# Autodesk Inventor assembly: Control Board Assembly
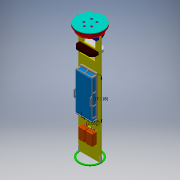
[picture p0: Inventor's stored thumbnail of the model, 180x180]
Saved by Autodesk Inventor 2016 (Build 200138000, 138)
## iProperties
Created: 2017-10-10
Part Number: Control Board Assembly
Document SubType Name: Assembly
Designer: Student
Author: Student
## Documents named in this file (21)
- C:\Users\Student\Documents\Derek Code and Projects\Autodesk\Control Board Assembly.iam
- C:\Users\Student\Documents\Derek Code and Projects\Autodesk\Control board Holder.ipt
- C:\Users\Student\Documents\Derek Code and Projects\Autodesk\Control Board.ipt
- C:\Users\Student\Documents\Derek Code and Projects\Autodesk\Control board Ring Holder.ipt
- C:\Users\Student\Documents\Derek Code and Projects\Autodesk\THE ACTUAL BACK O-RONG FITTING Connection to control board.ipt
- C:\Users\Student\Documents\Derek Code and Projects\Autodesk\Camera Mount.ipt
- C:\Users\Student\Documents\Derek Code and Projects\Autodesk\Camera.ipt
- C:\Users\Student\Documents\Derek Code and Projects\Autodesk\RPI.ipt
- C:\Users\Student\Documents\Derek Code and Projects\Autodesk\Arduino board with Sheild.ipt
- C:\Users\Student\Documents\Derek Code and Projects\Autodesk\Battery.ipt
- C:\Users\Student\Documents\Derek Code and Projects\Autodesk\Voltage Divider (Rough).ipt
- C:\Users\Student\Documents\Derek Code and Projects\Autodesk\Back Lens.ipt
- C:\Users\Student\Documents\Derek Code and Projects\Autodesk\Wire fitting End.ipt
- C:\Users\Student\Documents\Inventor\Content Center Files\R2016\en-US\BS 4183(7)\BS 4183 - M2.5 x 5(2) III.ipt
- C:\Users\Student\Documents\Inventor\Content Center Files\R2016\en-US\BS 4183(7)\BS 4183 - M3 x 5(2) III.ipt
- C:\Users\Student\Documents\Inventor\Content Center Files\R2016\en-US\BS 4183(7)\BS 4183 - M4 x 5(2) III.ipt
- C:\Users\Student\Documents\Derek Code and Projects\Autodesk\MEGA BATTERY MOUNT.ipt
- C:\Users\Student\Documents\Derek Code and Projects\Autodesk\Control Board Ring Slot Holder.ipt
- C:\Users\Student\Documents\Derek Code and Projects\Autodesk\LED Driver.ipt
- C:\Users\Student\Documents\Inventor\Content Center Files\R2016\en-US\CNS 3982 - AB\CNS 3982 - M4.2 x 9.5AB.ipt
- C:\Users\Student\Documents\Inventor\Content Center Files\R2016\en-US\CNS 3982 - AB\CNS 3982 - M2.9 x 6.5AB.ipt
## Components (56 placed, 20 different names)
1. Control board Holder:1 — Mate:36, Mate:37, Mate:38, Insert:13, Insert:14, Insert:15, Insert:36
2. Control board Holder:2 — Mate:34, Mate:35, Mate:39, Mate:40, Insert:10, Insert:11, Insert:12, Insert:37
3. Control Board:1 — Mate:29, Mate:30, Flush:1, Mate:34, Mate:35, Mate:36, Mate:37, Mate:43, Mate:46, Mate:47, Mate:48, Mate:51, Mate:53, Mate:54, Mate:55, Mate:56, Mate:57, Mate:58, Insert:8, Insert:9, Mate:72, Mate:73, Mate:74, Mate:80, Mate:81, Mate:82, Mate:83, Mate:84, Mate:85, Mate:87, Mate:88, Mate:89, Mate:90, Mate:91, Mate:92, Mate:93, Flush:2, Flush:3, Flush:4, Flush:5, Mate:94, Mate:95
4. Control board Ring Holder:1 — Mate:78, Mate:79, Mate:86
5. THE ACTUAL BACK O-RONG FITTING Connection to control board:1 — Mate:38, Mate:39, Mate:40, Mate:59, Mate:60, Mate:61
6. Camera Mount:1 — Mate:43, Mate:44, Mate:45, Insert:4, Mate:89, Mate:90, Insert:32, Insert:33, Insert:34, Insert:35
7. Camera:1 — Mate:44, Mate:45
8. RPI:1 — Mate:46, Mate:47, Mate:48
9. Arduino board with Sheild:1 — Mate:51, Mate:91, Mate:92, Mate:93, Insert:30, Insert:31
10. Voltage Divider (Rough):1 — Mate:53, Mate:54, Mate:58, Mate:96, Mate:97, Mate:98, Mate:99
11. Voltage Divider (Rough):2 — Mate:55, Mate:56, Mate:57
12. Back Lens:1 — Mate:59, Mate:60, Mate:61, Mate:62, Mate:63, Mate:64, Mate:65, Mate:66, Mate:67, Mate:68, Mate:69, Mate:70, Mate:71, Insert:16, Insert:17, Insert:18, Insert:19, Insert:20, Insert:21
13. Wire fitting End:1 — Mate:64, Mate:65
14. Wire fitting End:2 — Mate:62, Mate:63
15. Wire fitting End:3 — Mate:68, Mate:69
16. Wire fitting End:4 — Mate:70, Mate:71
17. Wire fitting End:5 — Mate:66, Mate:67
18. BS 4183 Slotted Pan Head Machine Screw - Metric M2.5 x 5:4 — Insert:4
19. BS 4183 Slotted Pan Head Machine Screw - Metric M4 x 5:1 — Insert:8
20. BS 4183 Slotted Pan Head Machine Screw - Metric M4 x 5:2 — Insert:9
21. BS 4183 Slotted Pan Head Machine Screw - Metric M2.5 x 5:5 — Insert:10
22. BS 4183 Slotted Pan Head Machine Screw - Metric M2.5 x 5:6 — Insert:11
23. BS 4183 Slotted Pan Head Machine Screw - Metric M3 x 5:4 — Insert:12
24. BS 4183 Slotted Pan Head Machine Screw - Metric M2.5 x 5:7 — Insert:13
25. BS 4183 Slotted Pan Head Machine Screw - Metric M3 x 5:5 — Insert:14
26. BS 4183 Slotted Pan Head Machine Screw - Metric M2.5 x 5:8 — Insert:15
27. BS 4183 Slotted Pan Head Machine Screw - Metric M2.5 x 5:9 — Insert:16
28. BS 4183 Slotted Pan Head Machine Screw - Metric M2.5 x 5:10 — Insert:17
29. BS 4183 Slotted Pan Head Machine Screw - Metric M2.5 x 5:11 — Insert:18
30. BS 4183 Slotted Pan Head Machine Screw - Metric M2.5 x 5:12 — Insert:19
31. BS 4183 Slotted Pan Head Machine Screw - Metric M2.5 x 5:13 — Insert:20
32. BS 4183 Slotted Pan Head Machine Screw - Metric M2.5 x 5:14 — Insert:21
33. MEGA BATTERY MOUNT:1 — Mate:72, Mate:73, Mate:74, Mate:75, Mate:76, Mate:77, Insert:26, Insert:27, Insert:28, Insert:29
34. Battery:1 — Mate:75, Mate:76, Mate:77
35. Control Board Ring Slot Holder:1 — Mate:78, Mate:81, Mate:82, Mate:84, Mate:87
36. Control Board Ring Slot Holder:2 — Mate:79, Mate:80, Mate:83, Mate:85, Mate:86, Mate:88
37. LED Driver:1 — Flush:2, Flush:5, Mate:95, Insert:22, Insert:23
38. LED Driver:2 — Flush:3, Flush:4, Mate:94, Insert:24, Insert:25
39. CNS 3982 - AB M4.2 x 9.5:1 — Insert:22
40. CNS 3982 - AB M4.2 x 9.5:2 — Insert:23
41. CNS 3982 - AB M4.2 x 9.5:3 — Insert:24
42. CNS 3982 - AB M4.2 x 9.5:4 — Insert:25
43. CNS 3982 - AB M2.9 x 6.5:1 — Insert:26
44. CNS 3982 - AB M2.9 x 6.5:2 — Insert:27
45. CNS 3982 - AB M2.9 x 6.5:3 — Insert:28
46. CNS 3982 - AB M2.9 x 6.5:4 — Insert:29
47. CNS 3982 - AB M4.2 x 9.5:5 — Mate:96, Mate:97
48. CNS 3982 - AB M4.2 x 9.5:6 — Mate:98, Mate:99
49. CNS 3982 - AB M2.9 x 6.5:5 — Insert:30
50. CNS 3982 - AB M2.9 x 6.5:6 — Insert:31
51. CNS 3982 - AB M2.9 x 6.5:7 — Insert:32
52. CNS 3982 - AB M2.9 x 6.5:8 — Insert:33
53. CNS 3982 - AB M2.9 x 6.5:9 — Insert:34
54. CNS 3982 - AB M2.9 x 6.5:10 — Insert:35
55. CNS 3982 - AB M2.9 x 6.5:11 — Insert:36
56. CNS 3982 - AB M2.9 x 6.5:12 — Insert:37
## Relationships (99: Mate 63, Insert 31, Flush 5)
- Mate:29: Control Board:1
- Mate:30: Control Board:1
- Flush:1: Control Board:1
- Mate:34: Control board Holder:2 ↔ Control Board:1
- Mate:35: Control board Holder:2 ↔ Control Board:1
- Mate:36: Control board Holder:1 ↔ Control Board:1
- Mate:37: Control board Holder:1 ↔ Control Board:1
- Mate:38: Control board Holder:1 ↔ THE ACTUAL BACK O-RONG FITTING Connection to control board:1
- Mate:39: Control board Holder:2 ↔ THE ACTUAL BACK O-RONG FITTING Connection to control board:1
- Mate:40: Control board Holder:2 ↔ THE ACTUAL BACK O-RONG FITTING Connection to control board:1
- Mate:43: Control Board:1 ↔ Camera Mount:1
- Mate:44: Camera Mount:1 ↔ Camera:1
- Mate:45: Camera Mount:1 ↔ Camera:1
- Mate:46: Control Board:1 ↔ RPI:1
- Mate:47: Control Board:1 ↔ RPI:1
- Mate:48: Control Board:1 ↔ RPI:1
- Mate:51: Control Board:1 ↔ Arduino board with Sheild:1
- Mate:53: Control Board:1 ↔ Voltage Divider (Rough):1
- Mate:54: Control Board:1 ↔ Voltage Divider (Rough):1
- Mate:55: Control Board:1 ↔ Voltage Divider (Rough):2
- Mate:56: Control Board:1 ↔ Voltage Divider (Rough):2
- Mate:57: Control Board:1 ↔ Voltage Divider (Rough):2
- Mate:58: Control Board:1 ↔ Voltage Divider (Rough):1
- Mate:59: THE ACTUAL BACK O-RONG FITTING Connection to control board:1 ↔ Back Lens:1
- Mate:60: THE ACTUAL BACK O-RONG FITTING Connection to control board:1 ↔ Back Lens:1
- Mate:61: THE ACTUAL BACK O-RONG FITTING Connection to control board:1 ↔ Back Lens:1
- Mate:62: Back Lens:1 ↔ Wire fitting End:2
- Mate:63: Back Lens:1 ↔ Wire fitting End:2
- Mate:64: Back Lens:1 ↔ Wire fitting End:1
- Mate:65: Back Lens:1 ↔ Wire fitting End:1
- Mate:66: Back Lens:1 ↔ Wire fitting End:5
- Mate:67: Back Lens:1 ↔ Wire fitting End:5
- Mate:68: Back Lens:1 ↔ Wire fitting End:3
- Mate:69: Back Lens:1 ↔ Wire fitting End:3
- Mate:70: Back Lens:1 ↔ Wire fitting End:4
- Mate:71: Back Lens:1 ↔ Wire fitting End:4
- Insert:4: Camera Mount:1 ↔ BS 4183 Slotted Pan Head Machine Screw - Metric M2.5 x 5:4
- Insert:8: Control Board:1 ↔ BS 4183 Slotted Pan Head Machine Screw - Metric M4 x 5:1
- Insert:9: Control Board:1 ↔ BS 4183 Slotted Pan Head Machine Screw - Metric M4 x 5:2
- Insert:10: Control board Holder:2 ↔ BS 4183 Slotted Pan Head Machine Screw - Metric M2.5 x 5:5
- Insert:11: Control board Holder:2 ↔ BS 4183 Slotted Pan Head Machine Screw - Metric M2.5 x 5:6
- Insert:12: Control board Holder:2 ↔ BS 4183 Slotted Pan Head Machine Screw - Metric M3 x 5:4
- Insert:13: Control board Holder:1 ↔ BS 4183 Slotted Pan Head Machine Screw - Metric M2.5 x 5:7
- Insert:14: Control board Holder:1 ↔ BS 4183 Slotted Pan Head Machine Screw - Metric M3 x 5:5
- Insert:15: Control board Holder:1 ↔ BS 4183 Slotted Pan Head Machine Screw - Metric M2.5 x 5:8
- Insert:16: Back Lens:1 ↔ BS 4183 Slotted Pan Head Machine Screw - Metric M2.5 x 5:9
- Insert:17: Back Lens:1 ↔ BS 4183 Slotted Pan Head Machine Screw - Metric M2.5 x 5:10
- Insert:18: Back Lens:1 ↔ BS 4183 Slotted Pan Head Machine Screw - Metric M2.5 x 5:11
- Insert:19: Back Lens:1 ↔ BS 4183 Slotted Pan Head Machine Screw - Metric M2.5 x 5:12
- Insert:20: Back Lens:1 ↔ BS 4183 Slotted Pan Head Machine Screw - Metric M2.5 x 5:13
- Insert:21: Back Lens:1 ↔ BS 4183 Slotted Pan Head Machine Screw - Metric M2.5 x 5:14
- Mate:72: Control Board:1 ↔ MEGA BATTERY MOUNT:1
- Mate:73: Control Board:1 ↔ MEGA BATTERY MOUNT:1
- Mate:74: Control Board:1 ↔ MEGA BATTERY MOUNT:1
- Mate:75: MEGA BATTERY MOUNT:1 ↔ Battery:1
- Mate:76: MEGA BATTERY MOUNT:1 ↔ Battery:1
- Mate:77: MEGA BATTERY MOUNT:1 ↔ Battery:1
- Mate:78: Control board Ring Holder:1 ↔ Control Board Ring Slot Holder:1
- Mate:79: Control board Ring Holder:1 ↔ Control Board Ring Slot Holder:2
- Mate:80: Control Board:1 ↔ Control Board Ring Slot Holder:2
- Mate:81: Control Board:1 ↔ Control Board Ring Slot Holder:1
- Mate:82: Control Board:1 ↔ Control Board Ring Slot Holder:1
- Mate:83: Control Board:1 ↔ Control Board Ring Slot Holder:2
- Mate:84: Control Board:1 ↔ Control Board Ring Slot Holder:1
- Mate:85: Control Board:1 ↔ Control Board Ring Slot Holder:2
- Mate:86: Control board Ring Holder:1 ↔ Control Board Ring Slot Holder:2
- Mate:87: Control Board:1 ↔ Control Board Ring Slot Holder:1
- Mate:88: Control Board:1 ↔ Control Board Ring Slot Holder:2
- Mate:89: Control Board:1 ↔ Camera Mount:1
- Mate:90: Control Board:1 ↔ Camera Mount:1
- Mate:91: Control Board:1 ↔ Arduino board with Sheild:1
- Mate:92: Control Board:1 ↔ Arduino board with Sheild:1
- Mate:93: Control Board:1 ↔ Arduino board with Sheild:1
- Flush:2 (-19.1516 mm): Control Board:1 ↔ LED Driver:1
- Flush:3 (17.5006 mm): Control Board:1 ↔ LED Driver:2
- Flush:4 (63.6778 mm): Control Board:1 ↔ LED Driver:2
- Flush:5 (63.6778 mm): Control Board:1 ↔ LED Driver:1
- Mate:94: Control Board:1 ↔ LED Driver:2
- Mate:95: Control Board:1 ↔ LED Driver:1
- Insert:22: LED Driver:1 ↔ CNS 3982 - AB M4.2 x 9.5:1
- Insert:23: LED Driver:1 ↔ CNS 3982 - AB M4.2 x 9.5:2
- Insert:24: LED Driver:2 ↔ CNS 3982 - AB M4.2 x 9.5:3
- Insert:25: LED Driver:2 ↔ CNS 3982 - AB M4.2 x 9.5:4
- Insert:26: MEGA BATTERY MOUNT:1 ↔ CNS 3982 - AB M2.9 x 6.5:1
- Insert:27: MEGA BATTERY MOUNT:1 ↔ CNS 3982 - AB M2.9 x 6.5:2
- Insert:28: MEGA BATTERY MOUNT:1 ↔ CNS 3982 - AB M2.9 x 6.5:3
- Insert:29: MEGA BATTERY MOUNT:1 ↔ CNS 3982 - AB M2.9 x 6.5:4
- Mate:96: Voltage Divider (Rough):1 ↔ CNS 3982 - AB M4.2 x 9.5:5
- Mate:97: Voltage Divider (Rough):1 ↔ CNS 3982 - AB M4.2 x 9.5:5
- Mate:98: Voltage Divider (Rough):1 ↔ CNS 3982 - AB M4.2 x 9.5:6
- Mate:99: Voltage Divider (Rough):1 ↔ CNS 3982 - AB M4.2 x 9.5:6
- Insert:30: Arduino board with Sheild:1 ↔ CNS 3982 - AB M2.9 x 6.5:5
- Insert:31: Arduino board with Sheild:1 ↔ CNS 3982 - AB M2.9 x 6.5:6
- Insert:32: Camera Mount:1 ↔ CNS 3982 - AB M2.9 x 6.5:7
- Insert:33: Camera Mount:1 ↔ CNS 3982 - AB M2.9 x 6.5:8
- Insert:34: Camera Mount:1 ↔ CNS 3982 - AB M2.9 x 6.5:9
- Insert:35: Camera Mount:1 ↔ CNS 3982 - AB M2.9 x 6.5:10
- Insert:36: Control board Holder:1 ↔ CNS 3982 - AB M2.9 x 6.5:11
- Insert:37: Control board Holder:2 ↔ CNS 3982 - AB M2.9 x 6.5:12
